# Autodesk Inventor assembly: ring assembly
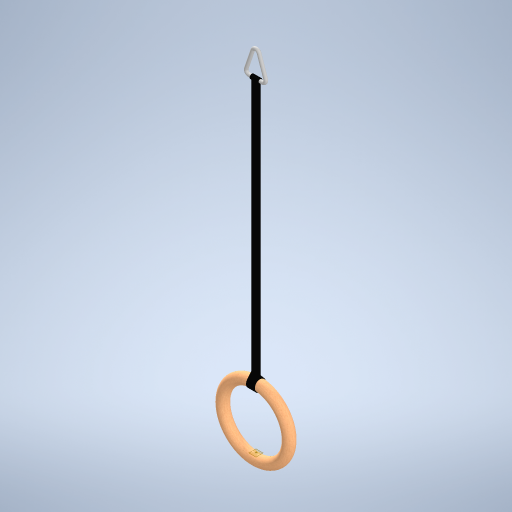
[picture p0: Inventor's stored thumbnail of the model, 512x512]
Saved by Autodesk Inventor 2024 (Build 280153000, 153)
## iProperties
Created: 2023-05-23
Part Number: ring assembly
Document SubType Name: Assembly
Designer: Patrick
Author: Patrick
## Documents named in this file (4)
- M:\Daten\Timeline\2023-05-22 Pull-Up Bar\cad\ring assembly.iam
- M:\Daten\Timeline\2023-05-22 Pull-Up Bar\cad\ring.ipt
- M:\Daten\Timeline\2023-05-22 Pull-Up Bar\cad\strap.ipt
- M:\Daten\Timeline\2023-05-22 Pull-Up Bar\cad\triange carabiner.ipt
## Components (3 placed, 3 different names)
1. ring:1 — Mate:7
2. strap:1 — Flush:3
3. triange carabiner:1 — Flush:2, Flush:4, Flush:5
## Relationships (9: Mate 5, Flush 4)
- [Mate]: ring:1 ↔ strap:1
- [Mate]: ring:1 ↔ strap:1
- [Mate] (100 mm): ring:1 ↔ strap:1
- [Mate]: strap:1 ↔ triange carabiner:1
- Flush:2: triange carabiner:1
- Mate:7: ring:1
- Flush:3: strap:1
- Flush:4: triange carabiner:1
- Flush:5: triange carabiner:1
